# Autodesk Inventor assembly: antenna_assembly_v2
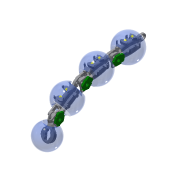
[picture p0: Inventor's stored thumbnail of the model, 180x180]
Saved by Autodesk Inventor 2017 (Build 210142000, 142)
## iProperties
Created: 2018-06-04
Part Number: antenna_assembly_v2
Document SubType Name: Assembly
Designer: Nic
Author: Nic
## Documents named in this file (7)
- C:\Users\Nic\Documents\Antenna\antenna_assembly_v2.iam
- C:\Users\Nic\Documents\Antenna\middle_segment_v2.ipt
- C:\Users\Nic\Documents\Antenna\sensor_pad.ipt
- C:\Users\Nic\Documents\Antenna\pizeo_sensor.ipt
- C:\Users\Nic\Documents\Antenna\end_segment_v2.ipt
- C:\Users\Nic\Documents\Antenna\encoder_coarse.ipt
- C:\Users\Nic\Documents\Antenna\end_pad.ipt
## Components (15 placed, 6 different names)
1. middle_segment_v2:3 — Insert:2, Insert:6, Flush:1, Mate:8
2. sensor_pad:3 — Flush:1, Mate:7
3. middle_segment_v2:2 — Insert:2, Insert:5, Flush:16, Insert:7, Mate:6
4. sensor_pad:2 — Flush:16, Mate:5
5. middle_segment_v2:1 — Insert:3, Insert:4, Flush:17, Insert:7, Mate:4
6. sensor_pad:1 — Flush:17, Mate:3
7. end_segment_v2:1 — Insert:3, Cylindrical:4, Flush:18, Mate:2
8. end_pad:1 — Flush:18, Mate:1
9. pizeo_sensor:1
10. pizeo_sensor:2
11. pizeo_sensor:3
12. pizeo_sensor:4 — Cylindrical:4
13. encoder_coarse:1 — Insert:4
14. encoder_coarse:2 — Insert:5
15. encoder_coarse:3 — Insert:6
## Relationships (19: Mate 8, Insert 6, Flush 4, CylindricalJoint 1)
- Insert:2 (2.5 mm): middle_segment_v2:3 ↔ middle_segment_v2:2
- Insert:3 (2.5 mm): middle_segment_v2:1 ↔ end_segment_v2:1
- Cylindrical:4: end_segment_v2:1 ↔ pizeo_sensor:4
- Insert:4: middle_segment_v2:1 ↔ encoder_coarse:1
- Insert:5: middle_segment_v2:2 ↔ encoder_coarse:2
- Insert:6: middle_segment_v2:3 ↔ encoder_coarse:3
- Flush:16 (1 mm): middle_segment_v2:2 ↔ sensor_pad:2
- Flush:17 (1 mm): middle_segment_v2:1 ↔ sensor_pad:1
- Flush:1 (1 mm): middle_segment_v2:3 ↔ sensor_pad:3
- Insert:7 (2.5 mm): middle_segment_v2:2 ↔ middle_segment_v2:1
- Flush:18: end_segment_v2:1 ↔ end_pad:1
- Mate:1: end_pad:1
- Mate:2: end_segment_v2:1
- Mate:3: sensor_pad:1
- Mate:4: middle_segment_v2:1
- Mate:5: sensor_pad:2
- Mate:6: middle_segment_v2:2
- Mate:7: sensor_pad:3
- Mate:8: middle_segment_v2:3
